# Autodesk Inventor assembly: main
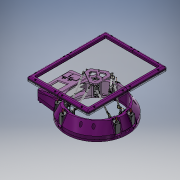
[picture p0: Inventor's stored thumbnail of the model, 180x180]
Saved by Autodesk Inventor 2017 (Build 210142000, 142)
## iProperties
Part Number: main
Material: Ogólny
Document SubType Name: Assembly
Designer: Speed King
Mass: 2741.05 g
Surface Area: 7362.62 cm^2
Volume: 2457.67 cm^3
Density: 1.1153 g/cm^3
Author: Speed King
## Documents named in this file (11)
- C:\Users\Speed King\Documents\My Inventor\GrabCAD\Technical Informatics\CAD\model\main.iam
- C:\Users\Speed King\Documents\My Inventor\GrabCAD\Technical Informatics\CAD\model\section_ground.iam
- C:\Users\Speed King\Documents\My Inventor\GrabCAD\Technical Informatics\CAD\model\section_lever.iam
- C:\Users\Speed King\Documents\My Inventor\GrabCAD\Technical Informatics\CAD\model\section_rod.iam
- C:\Users\Speed King\Documents\My Inventor\GrabCAD\Technical Informatics\CAD\model\section_upper.iam
- C:\Users\Speed King\Documents\My Inventor\GrabCAD\Technical Informatics\CAD\model\stm32f429.ipt
- C:\Users\Speed King\Documents\My Inventor\GrabCAD\Technical Informatics\CAD\model\bolts\Design Accelerator\Połączenie gwintowe1.iam
- C:\Users\Speed King\Documents\My Inventor\GrabCAD\Technical Informatics\CAD\model\pcb.ipt
- C:\Users\Speed King\Documents\My Inventor\GrabCAD\Technical Informatics\CAD\model\housing_ground.ipt
- C:\Users\Speed King\Documents\My Inventor\GrabCAD\Technical Informatics\CAD\model\housing_cover.ipt
- C:\Users\Speed King\Documents\My Inventor\GrabCAD\Technical Informatics\CAD\model\housing_legs.ipt
## Components (21 placed, 10 different names)
1. section_upper:1 [sub-assembly] — Zestawiający:19, Zestawiający:20, Zestawiający:21, Zestawiający:22, Zestawiający:23, Zestawiający:24, Kąt:15, Kąt:16
2. section_ground:1 [sub-assembly] — Zestawiający:1, Zestawiający:3, Zestawiający:5, Zestawiający:7, Zestawiający:9, Równoległy:26, Równoległy:27, Zestawiający:29, Zestawiający:30, Zestawiający:31, Zestawiający:32, Zestawiający:33, Zestawiający:34, Zestawiający:35, Zestawiający:36, Kąt:7, Kąt:8, Kąt:9, Kąt:10, Kąt:11, Kąt:12, Kąt:15, Zestawiający:39, Zestawiający:40, Równoległy:32, Równoległy:33, Zestawiający:45, Zestawiający:46, Zestawiający:51
3. section_lever:1 [sub-assembly] — Zestawiający:15, Kąt:12, Zestawiający:30, Zestawiający:31
4. section_rod:1 [sub-assembly] — Zestawiający:15, Zestawiający:21
5. section_lever:2 [sub-assembly] — Zestawiający:1, Zestawiający:14, Zestawiający:32, Kąt:7
6. section_rod:2 [sub-assembly] — Zestawiający:14, Zestawiający:20
7. section_lever:3 [sub-assembly] — Zestawiający:3, Zestawiający:13, Kąt:8, Zestawiający:33
8. section_rod:3 [sub-assembly] — Zestawiający:13, Zestawiający:19
9. section_lever:4 [sub-assembly] — Zestawiający:5, Zestawiający:18, Kąt:9, Zestawiający:34
10. section_rod:4 [sub-assembly] — Zestawiający:18, Zestawiający:24
11. section_lever:5 [sub-assembly] — Zestawiający:7, Zestawiający:17, Kąt:10, Zestawiający:35
12. section_rod:5 [sub-assembly] — Zestawiający:17, Zestawiający:23
13. section_lever:6 [sub-assembly] — Zestawiający:9, Zestawiający:16, Kąt:11, Zestawiający:36
14. section_rod:6 [sub-assembly] — Zestawiający:16, Zestawiający:22
15. Połączenie gwintowe:1 [sub-assembly] — Zestawiający:39, Zestawiający:40
16. stm32f429:1 — Zestawiający:58, Równoległy:43, Równoległy:44
17. pcb:1 — Zestawiający:48, Zestawiający:53, Zestawiający:58, Równoległy:43, Równoległy:44
18. housing_legs:1 — Zestawiający:54, Zestawiający:56
19. housing_legs:2 — Zestawiający:55, Zestawiający:57
20. housing_ground:1 — Równoległy:32, Równoległy:33, Zestawiający:45, Zestawiający:46, Równoległy:39, Zestawiający:52, Zestawiający:53, Zestawiający:54, Zestawiający:55, Zestawiający:56, Zestawiający:57
21. housing_cover:1 — Zestawiający:51, Równoległy:39, Zestawiający:52
## Relationships (53: Mate 38, Angle 8, Flush 7)
- Zestawiający:1 [Mate]: section_ground:1 ↔ section_lever:2
- Zestawiający:3 [Mate]: section_ground:1 ↔ section_lever:3
- Zestawiający:5 [Mate]: section_ground:1 ↔ section_lever:4
- Zestawiający:7 [Mate]: section_ground:1 ↔ section_lever:5
- Zestawiający:9 [Mate]: section_ground:1 ↔ section_lever:6
- Zestawiający:13 [Mate]: section_lever:3 ↔ section_rod:3
- Zestawiający:14 [Mate]: section_lever:2 ↔ section_rod:2
- Zestawiający:15 [Mate]: section_lever:1 ↔ section_rod:1
- Zestawiający:16 [Mate]: section_lever:6 ↔ section_rod:6
- Zestawiający:17 [Mate]: section_lever:5 ↔ section_rod:5
- Zestawiający:18 [Mate]: section_lever:4 ↔ section_rod:4
- Zestawiający:19 [Mate]: section_upper:1 ↔ section_rod:3
- Zestawiający:20 [Mate]: section_upper:1 ↔ section_rod:2
- Zestawiający:21 [Mate]: section_upper:1 ↔ section_rod:1
- Zestawiający:22 [Mate]: section_upper:1 ↔ section_rod:6
- Zestawiający:23 [Mate]: section_upper:1 ↔ section_rod:5
- Zestawiający:24 [Mate]: section_upper:1 ↔ section_rod:4
- Równoległy:26 [Flush]: section_ground:1
- Równoległy:27 [Flush]: section_ground:1
- Zestawiający:29 [Mate]: section_ground:1
- Zestawiający:30 [Mate]: section_ground:1 ↔ section_lever:1
- Zestawiający:31 [Mate]: section_ground:1 ↔ section_lever:1
- Zestawiający:32 [Mate]: section_ground:1 ↔ section_lever:2
- Zestawiający:33 [Mate]: section_ground:1 ↔ section_lever:3
- Zestawiający:34 [Mate]: section_ground:1 ↔ section_lever:4
- Zestawiający:35 [Mate]: section_ground:1 ↔ section_lever:5
- Zestawiający:36 [Mate]: section_ground:1 ↔ section_lever:6
- Kąt:7 [Angle] (0 deg): section_ground:1 ↔ section_lever:2
- Kąt:8 [Angle] (180 deg): section_ground:1 ↔ section_lever:3
- Kąt:9 [Angle] (0 deg): section_ground:1 ↔ section_lever:4
- Kąt:10 [Angle] (180 deg): section_ground:1 ↔ section_lever:5
- Kąt:11 [Angle] (0 deg): section_ground:1 ↔ section_lever:6
- Kąt:12 [Angle] (180 deg): section_ground:1 ↔ section_lever:1
- Kąt:15 [Angle] (0 deg): section_upper:1 ↔ section_ground:1
- Kąt:16 [Angle] (180 deg): section_upper:1
- Zestawiający:39 [Mate]: section_ground:1 ↔ Połączenie gwintowe:1
- Zestawiający:40 [Mate]: section_ground:1 ↔ Połączenie gwintowe:1
- Równoległy:32 [Flush]: section_ground:1 ↔ housing_ground:1
- Równoległy:33 [Flush]: section_ground:1 ↔ housing_ground:1
- Zestawiający:45 [Mate]: section_ground:1 ↔ housing_ground:1
- Zestawiający:46 [Mate]: section_ground:1 ↔ housing_ground:1
- Zestawiający:48 [Mate]: pcb:1
- Zestawiający:51 [Mate]: section_ground:1 ↔ housing_cover:1
- Równoległy:39 [Flush]: housing_ground:1 ↔ housing_cover:1
- Zestawiający:52 [Mate]: housing_ground:1 ↔ housing_cover:1
- Zestawiający:53 [Mate]: pcb:1 ↔ housing_ground:1
- Zestawiający:54 [Mate]: housing_legs:1 ↔ housing_ground:1
- Zestawiający:55 [Mate]: housing_legs:2 ↔ housing_ground:1
- Zestawiający:56 [Mate]: housing_legs:1 ↔ housing_ground:1
- Zestawiający:57 [Mate]: housing_legs:2 ↔ housing_ground:1
- Zestawiający:58 [Mate] (-15 mm): stm32f429:1 ↔ pcb:1
- Równoległy:43 [Flush]: stm32f429:1 ↔ pcb:1
- Równoległy:44 [Flush] (9 mm): stm32f429:1 ↔ pcb:1
